# Autodesk Inventor assembly: przegub_5
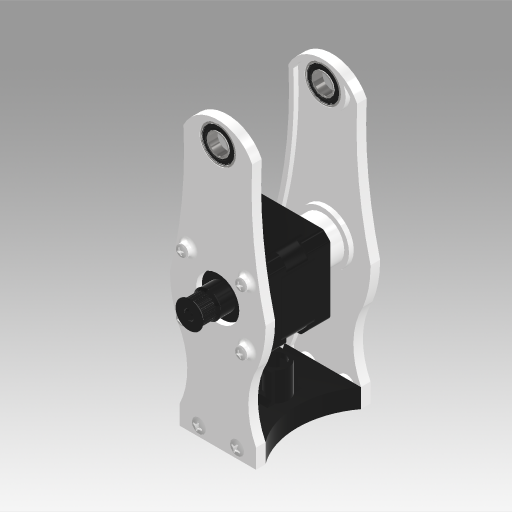
[picture p0: Inventor's stored thumbnail of the model, 512x512]
Saved by Autodesk Inventor 2024.3 (Build 283343000, 343)
## iProperties
Created: 2025-10-11
Part Number: przegub_5
Document SubType Name: Assembly
Designer: User
Mass: 105.034 g
Surface Area: 680.617 cm^2
Volume: 105.034 cm^3
Density: 1 g/cm^3
Author: User
## Documents named in this file (12)
- C:\Users\Duszy\Desktop\Dummy_v2\Model\Model\przegub_5\przegub_5.iam
- C:\Users\Duszy\Desktop\Dummy_v2\Model\Model\przegub_5\17HS13-0404S.ipt
- C:\Users\Duszy\Desktop\Dummy_v2\Model\Model\przegub_5\20_zb_wal.ipt
- C:\Users\Duszy\Desktop\Dummy_v2\Model\Model\przegub_5\OS_5+6_ramie1.ipt
- C:\Users\Duszy\Desktop\Dummy_v2\Model\Model\przegub_5\OS_5+6_ramie1_clean.ipt
- C:\Users\Duszy\Desktop\Dummy_v2\Model\Model\przegub_5\OS_REKA.ipt
- C:\Users\Duszy\Desktop\Dummy_v2\Model\Model z feedback\przegub_3\m4-10mm.ipt
- C:\Users\Duszy\Desktop\Dummy_v2\Model\Model\przegub_5\m3-10mm.ipt
- C:\Users\Duszy\Desktop\Dummy_v2\Model\Model\przegub_5\94459A150_Heat-Set Inserts for Plastic.ipt
- C:\Users\Duszy\Desktop\Dummy_v2\Model\Model z feedback\przegub_3\m4-10mm_MIR.ipt
- C:\Users\Duszy\Desktop\Dummy_v2\Model\Model\przegub_5\94459A150_Heat-Set Inserts for Plastic_MIR.ipt
- C:\Users\Duszy\Desktop\Dummy_v2\Model\Model\5972K275_Ball Bearing.ipt
## Components (19 placed, 11 different names)
1. 17HS13-0404S:1 — Obrotowe:7, Obrotowe:8, Obrotowe:10
2. 20_zb_wal:1 — Obrotowe:7
3. OS_5+6_ramie1:1 — Obrotowe:6, Obrotowe:11
4. OS_5+6_ramie1_clean:1 — Obrotowe:2, Obrotowe:8, Obrotowe:9, Obrotowe:12
5. OS_REKA:1 — Obrotowe:1, Obrotowe:5, Równoległe:1, Obrotowe:6, Obrotowe:9
6. m4-10mm:1 — Obrotowe:3
7. 94459A150_Heat-Set Inserts for Plastic:1 — Obrotowe:1, Obrotowe:2, Obrotowe:3
8. m4-10mm:3 — Obrotowe:4
9. 94459A150_Heat-Set Inserts for Plastic:3 — Obrotowe:4, Obrotowe:5
10. m4-10mm_MIR:1
11. 94459A150_Heat-Set Inserts for Plastic_MIR:1
12. m4-10mm_MIR:2
13. 94459A150_Heat-Set Inserts for Plastic_MIR:2
14. 5972K275_Ball Bearing:1 — Obrotowe:12
15. 5972K275_Ball Bearing:2 — Obrotowe:11
16. m3-10mm:1 — Obrotowe:10
17. m3-10mm:2
18. m3-10mm:3
19. m3-10mm:4
## Component patterns: (4 elements, first: m3-10mm:1)
## Relationships (13: RevoluteJoint 12, Flush 1)
- Obrotowe:1 [RevoluteJoint]: OS_REKA:1 ↔ 94459A150_Heat-Set Inserts for Plastic:1
- Obrotowe:2 [RevoluteJoint]: OS_5+6_ramie1_clean:1 ↔ 94459A150_Heat-Set Inserts for Plastic:1
- Obrotowe:3 [RevoluteJoint] (-5 mm): m4-10mm:1 ↔ 94459A150_Heat-Set Inserts for Plastic:1
- Obrotowe:4 [RevoluteJoint] (-5 mm): m4-10mm:3 ↔ 94459A150_Heat-Set Inserts for Plastic:3
- Obrotowe:5 [RevoluteJoint]: OS_REKA:1 ↔ 94459A150_Heat-Set Inserts for Plastic:3
- Równoległe:1 [Flush] (-25 mm): OS_REKA:1
- Obrotowe:6 [RevoluteJoint]: OS_5+6_ramie1:1 ↔ OS_REKA:1
- Obrotowe:7 [RevoluteJoint]: 17HS13-0404S:1 ↔ 20_zb_wal:1
- Obrotowe:8 [RevoluteJoint]: 17HS13-0404S:1 ↔ OS_5+6_ramie1_clean:1
- Obrotowe:9 [RevoluteJoint]: OS_5+6_ramie1_clean:1 ↔ OS_REKA:1
- Obrotowe:10 [RevoluteJoint] (2 mm): 17HS13-0404S:1 ↔ m3-10mm:1
- Obrotowe:11 [RevoluteJoint] (-4.8 mm): OS_5+6_ramie1:1 ↔ 5972K275_Ball Bearing:2
- Obrotowe:12 [RevoluteJoint] (-2.5 mm): OS_5+6_ramie1_clean:1 ↔ 5972K275_Ball Bearing:1
